# Autodesk Inventor assembly: Power Board
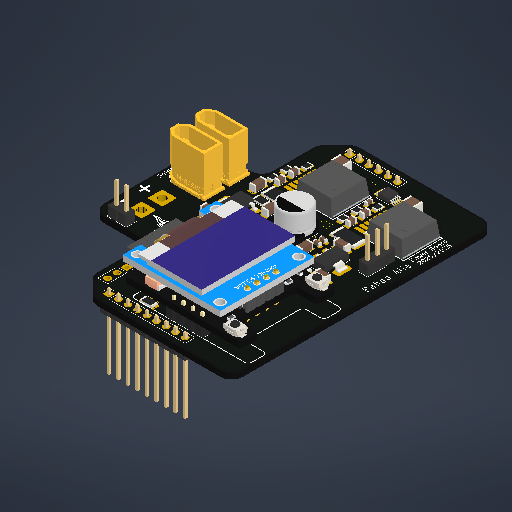
[picture p0: Inventor's stored thumbnail of the model, 512x512]
Saved by Autodesk Inventor 2026.1 (Build 301233020, 233B)
## iProperties
Company: Kicad
Created: 2026-05-17
Part Number: Power Board
Description: KiCad electronic assembly
Document SubType Name: Assembly
Designer: Bahaa
Authority: Unknown
Mass: 16.4413 g
Surface Area: 334.563 cm^2
Volume: 12.2517 cm^3
Density: 1.34196 g/cm^3
Sending System: KiCad to STEP converter
Preprocessor: Open CASCADE STEP processor 7.9
Title: Power Board.step
Author: Pcbnew
## Documents named in this file (28)
- C:\Users\Bahaa\Nextcloud2\CAD\25-26\V2\Boards\Power Board\Power Board\Power Board.iam
- C:\Users\Bahaa\Nextcloud2\CAD\25-26\V2\Boards\Power Board\Power Board\PRT-10158_PinHeader_1x09_P2.54mm_Vertical.ipt
- C:\Users\Bahaa\Nextcloud2\CAD\25-26\V2\Boards\Power Board\Power Board\R_0805_2012Metric.ipt
- C:\Users\Bahaa\Nextcloud2\CAD\25-26\V2\Boards\Power Board\Power Board\C_0805_2012Metric.ipt
- C:\Users\Bahaa\Nextcloud2\CAD\25-26\V2\Boards\Power Board\Power Board\NVRGS042N04CLT1G.iam
- C:\Users\Bahaa\Nextcloud2\CAD\25-26\V2\Boards\Power Board\Power Board\C_1206_3216Metric.ipt
- C:\Users\Bahaa\Nextcloud2\CAD\25-26\V2\Boards\Power Board\Power Board\R_2512_6332Metric.ipt
- C:\Users\Bahaa\Nextcloud2\CAD\25-26\V2\Boards\Power Board\Power Board\MAGI_C-VDRM_TO263-7EP_171032401.ipt
- C:\Users\Bahaa\Nextcloud2\CAD\25-26\V2\Boards\Power Board\Power Board\C_0603_1608Metric.ipt
- C:\Users\Bahaa\Nextcloud2\CAD\25-26\V2\Boards\Power Board\Power Board\C_1210_3225Metric.ipt
- C:\Users\Bahaa\Nextcloud2\CAD\25-26\V2\Boards\Power Board\Power Board\SOT-223.ipt
- C:\Users\Bahaa\Nextcloud2\CAD\25-26\V2\Boards\Power Board\Power Board\XT30U v1.ipt
- C:\Users\Bahaa\Nextcloud2\CAD\25-26\V2\Boards\Power Board\Power Board\EEE-FP1C221AL.iam
- C:\Users\Bahaa\Nextcloud2\CAD\25-26\V2\Boards\Power Board\Power Board\R_1206_3216Metric.ipt
- C:\Users\Bahaa\Nextcloud2\CAD\25-26\V2\Boards\Power Board\Power Board\PRT-10158_PinHeader_1x06_P2.54mm_Vertical.ipt
- C:\Users\Bahaa\Nextcloud2\CAD\25-26\V2\Boards\Power Board\Power Board\PinHeader_1x02_P2.54mm_Vertical.ipt
- C:\Users\Bahaa\Nextcloud2\CAD\25-26\V2\Boards\Power Board\Power Board\R_0603_1608Metric.ipt
- C:\Users\Bahaa\Nextcloud2\CAD\25-26\V2\Boards\Power Board\Power Board\PinHeader_1x03_P2.54mm_Vertical.ipt
- C:\Users\Bahaa\Nextcloud2\CAD\25-26\V2\Boards\Power Board\Power Board\TSSOP-10_3x3mm_P0.5mm.ipt
- C:\Users\Bahaa\Nextcloud2\CAD\25-26\V2\Boards\Power Board\Power Board\Same_Sky_CEM-1212S.ipt
- C:\Users\Bahaa\Nextcloud2\CAD\25-26\V2\Boards\Power Board\Power Board\TO-252-2.iam
- C:\Users\Bahaa\Nextcloud2\CAD\25-26\V2\Boards\Power Board\Power Board\Power Board_copper.ipt
- C:\Users\Bahaa\Nextcloud2\CAD\25-26\V2\Boards\Power Board\Power Board\Power Board_pad.ipt
- C:\Users\Bahaa\Nextcloud2\CAD\25-26\V2\Boards\Power Board\Power Board\Power Board_via.ipt
- C:\Users\Bahaa\Nextcloud2\CAD\25-26\V2\Boards\Power Board\Power Board\Power Board_silkscreen.ipt
- C:\Users\Bahaa\Nextcloud2\CAD\25-26\V2\Boards\Power Board\Power Board\Power Board_silkscreen_1.ipt
- C:\Users\Bahaa\Nextcloud2\CAD\25-26\V2\Boards\Power Board\Power Board\Power Board_PCB.ipt
- C:\Users\Bahaa\Nextcloud2\CAD\25-26\V2\Parts\modul_v3\hg_modul_3d.iam
## Components (56 placed, 56 different names)
1. 1
2. 2
3. 3
4. 7 [sub-assembly]
5. 8
6. 9
7. 10
8. 11
9. 12
10. 13
11. 14
12. 15
13. 16
14. 17
15. 22 [sub-assembly]
16. 23
17. 24
18. 25
19. 26
20. 27
21. 28 — Mate:3, Flush:1, Mate:4
22. 29
23. 30
24. 31
25. 32
26. 33
27. 34
28. 35
29. 36
30. 37
31. 38
32. 39
33. 40
34. 41
35. 43
36. 44
37. 45
38. 46
39. 47
40. 48
41. 49
42. 50
43. 51
44. 52
45. 54 [sub-assembly]
46. 55
47. 56
48. 57
49. 58
50. 59 — Mate:1, Mate:3
51. 60 — Mate:4
52. 61
53. 62 — Mate:2
54. 63
55. 64 — Flush:1
56. hg_modul_3d:1 [sub-assembly] — Mate:1, Mate:2
## Relationships (5: Mate 4, Flush 1)
- Mate:1: 59 ↔ hg_modul_3d:1
- Mate:2 (0.1 mm): 62 ↔ hg_modul_3d:1
- Mate:3: 28 ↔ 59
- Flush:1 (0.49 mm): 28 ↔ 64
- Mate:4 (0.5275 mm): 28 ↔ 60
